# Autodesk Inventor assembly: Gearbox
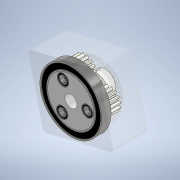
[picture p0: Inventor's stored thumbnail of the model, 180x180]
Saved by Autodesk Inventor 2022 (Build 260153000, 153)
## iProperties
Created: 2022-08-10
Part Number: Gearbox
Document SubType Name: Assembly
Designer: Nick
Author: Nick
## Documents named in this file (7)
- Y:\Projects\BattleBot\Gearbox.iam
- Y:\Projects\BattleBot\Gear Ring.ipt
- Y:\Projects\BattleBot\Planet Gear.ipt
- Y:\Projects\BattleBot\Sun Gear.ipt
- Y:\Projects\BattleBot\Carrier.ipt
- Y:\Projects\BattleBot\MR95ZZ Bearing.ipt
- Y:\Projects\BattleBot\6807 Bearing.ipt
## Components (13 placed, 6 different names)
1. Gear Ring:1 — Mate:4, Insert:13, Insert:15
2. Planet Gear:1 — Insert:6
3. Sun Gear:1 — Insert:15
4. Planet Gear:2 — Insert:7
5. Planet Gear:3 — Insert:8
6. MR95ZZ Bearing:1 — Insert:6, Insert:9
7. Carrier:1 — Insert:9, Insert:10, Insert:11, Mate:4, Insert:14, Insert:16, Insert:17, Insert:18
8. MR95ZZ Bearing:2 — Insert:8, Insert:10
9. MR95ZZ Bearing:4 — Insert:7, Insert:11
10. 6807 Bearing:1 — Insert:13, Insert:14
11. MR95ZZ Bearing:5 — Insert:18
12. MR95ZZ Bearing:6 — Insert:17
13. MR95ZZ Bearing:7 — Insert:16
## Relationships (13: Insert 12, Mate 1)
- Insert:6: Planet Gear:1 ↔ MR95ZZ Bearing:1
- Insert:7: Planet Gear:2 ↔ MR95ZZ Bearing:4
- Insert:8: Planet Gear:3 ↔ MR95ZZ Bearing:2
- Insert:9: MR95ZZ Bearing:1 ↔ Carrier:1
- Insert:10: Carrier:1 ↔ MR95ZZ Bearing:2
- Insert:11: Carrier:1 ↔ MR95ZZ Bearing:4
- Mate:4: Gear Ring:1 ↔ Carrier:1
- Insert:13: Gear Ring:1 ↔ 6807 Bearing:1
- Insert:14: Carrier:1 ↔ 6807 Bearing:1
- Insert:15: Gear Ring:1 ↔ Sun Gear:1
- Insert:16: Carrier:1 ↔ MR95ZZ Bearing:7
- Insert:17: Carrier:1 ↔ MR95ZZ Bearing:6
- Insert:18: Carrier:1 ↔ MR95ZZ Bearing:5
